# Autodesk Inventor assembly: Assemblage_partie_haute_étage
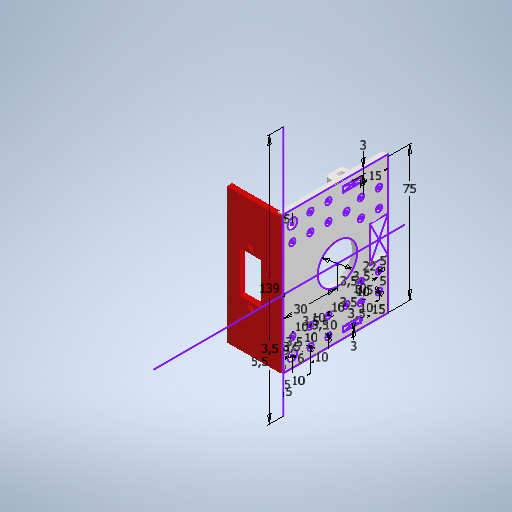
[picture p0: Inventor's stored thumbnail of the model, 512x512]
Saved by Autodesk Inventor 2025.1 (Build 291241000, 241)
## iProperties
Created: 2024-11-30
Part Number: Assemblage_partie_haute_étage
Document SubType Name: Assembly
Designer: yasmi
Author: yasmi
## Documents named in this file (3)
- C:\Users\yasmi\Desktop\PAMI-CdR-2025-main\PAMI-CdR-2025-main\Modeles_3D\Modifications\étage_BAU_et_étage_devant.iam
- C:\Users\yasmi\Desktop\PAMI-CdR-2025-main\PAMI-CdR-2025-main\Modeles_3D\Modifications\étage_devant.ipt
- C:\Users\yasmi\Desktop\PAMI-CdR-2025-main\PAMI-CdR-2025-main\Modeles_3D\Modifications\étage_BAU.ipt
## Components (2 placed, 2 different names)
1. étage_devant:1 — Rigide:3
2. étage_BAU:1 — Rigide:3
## Relationships (1: WeldJoint 1)
- Rigide:3 [WeldJoint]: étage_devant:1 ↔ étage_BAU:1
